# Autodesk Inventor assembly: jackAssembly
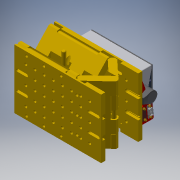
[picture p0: Inventor's stored thumbnail of the model, 180x180]
Saved by Autodesk Inventor 2016 (Build 200138000, 138)
## iProperties
Created: 2016-10-04
Part Number: jackAssembly
Document SubType Name: Assembly
Designer: sims01
Author: sims01
## Documents named in this file (5)
- H:\Documents\LSFM_3\setup\mechanical\design\lsfm3_mechDesign\jackAssembly.iam
- H:\Documents\LSFM_3\setup\mechanical\design\lsfm3_mechDesign\newportHighLoadJack.ipt
- H:\Documents\LSFM_3\setup\mechanical\design\lsfm3_mechDesign\piStage_Z.ipt
- H:\Documents\LSFM_3\setup\mechanical\design\lsfm3_mechDesign\zStackJackAttach_piece1.ipt
- H:\Documents\LSFM_3\setup\mechanical\design\lsfm3_mechDesign\zStackJackAttach_piece2.ipt
## Components (4 placed, 4 different names)
1. newportHighLoadJack:1 — Rigid:1, Rigid:2
2. piStage_Z:2 — Rigid:3
3. zStackJackAttach_piece1:1 — Rigid:1, Rigid:3
4. zStackJackAttach_piece2:1 — Rigid:2
## Relationships (3: WeldJoint 3)
- Rigid:1 [WeldJoint]: newportHighLoadJack:1 ↔ zStackJackAttach_piece1:1
- Rigid:2 [WeldJoint]: newportHighLoadJack:1 ↔ zStackJackAttach_piece2:1
- Rigid:3 [WeldJoint]: piStage_Z:2 ↔ zStackJackAttach_piece1:1
